# Autodesk Inventor assembly: tower_MIR
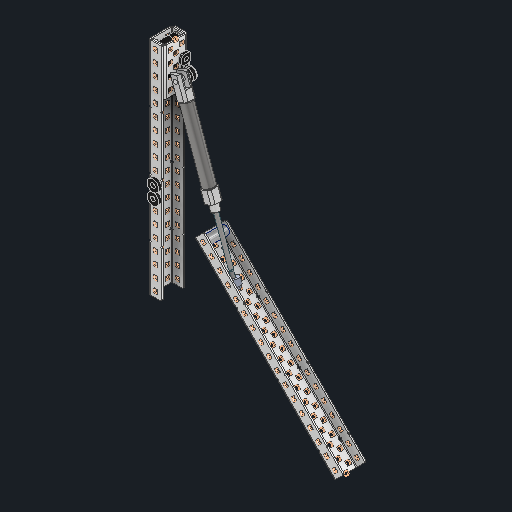
[picture p0: Inventor's stored thumbnail of the model, 512x512]
Saved by Autodesk Inventor 2024 (Build 280153000, 153)
## iProperties
Created: 2024-01-16
Part Number: tower_MIR
Document SubType Name: Assembly
Designer: Averey Ku
Author: avere
## Documents named in this file (16)
- D:\vex_robotics\hardware\cad\zoomba_v0.3\arm\tower_MIR.iam
- D:\vex_robotics\hardware\cad\zoomba_v0.3\arm\Alu C 1x2x1x19_MIR.ipt
- D:\vex_robotics\hardware\cad\zoomba_v0.3\arm\Alu C 1x2x1x4_MIR.ipt
- D:\vex_robotics\hardware\cad\VEX-CAD-Inventor-1.41\Motion\Spacers\Spacer Nylon .500 OD\NSpacer Black .500 OD x .125.ipt
- D:\vex_robotics\hardware\cad\VEX-CAD-Inventor-1.41\Motion\Spacers\Spacer Nylon .500 OD.ipt
- D:\vex_robotics\hardware\cad\zoomba_v0.3\arm\LS Pillow Bearing Block_MIR.ipt
- D:\vex_robotics\hardware\cad\VEX-CAD-Inventor-1.41\Motion\Spacers\Spacer Nylon .375 OD\NSpacer .375 OD x .250.ipt
- D:\vex_robotics\hardware\cad\VEX-CAD-Inventor-1.41\Motion\Spacers\Spacer Nylon .375 OD.ipt
- D:\vex_robotics\hardware\cad\VEX-CAD-Inventor-1.41\Motion\Spacers\Spacer Nylon .375 OD\NSpacer .375 OD x .500.ipt
- D:\vex_robotics\hardware\cad\VEX-CAD-Inventor-1.41\Motion\Spacers\Washer Steel\SWasher .375 OD x .062500.ipt
- D:\vex_robotics\hardware\cad\VEX-CAD-Inventor-1.41\Motion\Spacers\Washer Steel.ipt
- D:\vex_robotics\hardware\cad\zoomba_v0.3\arm\Double Acting Piston_MIR.iam
- D:\vex_robotics\hardware\cad\zoomba_v0.3\arm\Alu C 1x2x1x17_MIR.ipt
- D:\vex_robotics\hardware\cad\zoomba_v0.3\arm\Shaft Collar No Screw_MIR.ipt
- D:\vex_robotics\hardware\cad\zoomba_v0.3\arm\Piston Nut_MIR.ipt
- D:\vex_robotics\hardware\cad\zoomba_v0.3\arm\.375 OD Aluminum Spacer 0.875_MIR.ipt
## Components (13 placed, 12 different names)
1. Alu C 1x2x1x19_MIR:1 — Mate:1, Insert:1, Insert:4, Insert:3, Angle:1
2. Alu C 1x2x1x4_MIR:1 — Mate:1, Insert:1, Mate:2, Insert:5, Insert:8
3. NSpacer Black .500 OD x .125:1 — Insert:4
4. NSpacer Black .500 OD x .125:2 — Insert:3
5. LS Pillow Bearing Block_MIR:1 — Mate:2, Insert:5, Insert:9
6. NSpacer .375 OD x .250:1 — Insert:7, Insert:6
7. NSpacer .375 OD x .500:2 — Insert:8, Insert:7
8. SWasher .375 OD x .062500:1 — Insert:6
9. Double Acting Piston_MIR:1 [sub-assembly] — Insert:9, Insert:11
10. Alu C 1x2x1x17_MIR:1 — Angle:1, Mate:3, Insert:12
11. Shaft Collar No Screw_MIR:1 — Mate:3, Insert:10
12. Piston Nut_MIR:1 — Insert:11, Insert:10
13. .375 OD Aluminum Spacer 0.875_MIR:1 — Insert:12
## Relationships (15: Insert 11, Mate 3, Angle 1)
- Mate:1: Alu C 1x2x1x19_MIR:1 ↔ Alu C 1x2x1x4_MIR:1
- Insert:1: Alu C 1x2x1x19_MIR:1 ↔ Alu C 1x2x1x4_MIR:1
- Insert:4: Alu C 1x2x1x19_MIR:1 ↔ NSpacer Black .500 OD x .125:1
- Insert:3: Alu C 1x2x1x19_MIR:1 ↔ NSpacer Black .500 OD x .125:2
- Mate:2: Alu C 1x2x1x4_MIR:1 ↔ LS Pillow Bearing Block_MIR:1
- Insert:5 (1.5875 mm): Alu C 1x2x1x4_MIR:1 ↔ LS Pillow Bearing Block_MIR:1
- Insert:8: Alu C 1x2x1x4_MIR:1 ↔ NSpacer .375 OD x .500:2
- Insert:7: NSpacer .375 OD x .250:1 ↔ NSpacer .375 OD x .500:2
- Insert:6: NSpacer .375 OD x .250:1 ↔ SWasher .375 OD x .062500:1
- Insert:9: LS Pillow Bearing Block_MIR:1 ↔ Double Acting Piston_MIR:1
- Angle:1 (0 deg): Alu C 1x2x1x19_MIR:1 ↔ Alu C 1x2x1x17_MIR:1
- Mate:3: Alu C 1x2x1x17_MIR:1 ↔ Shaft Collar No Screw_MIR:1
- Insert:11: Double Acting Piston_MIR:1 ↔ Piston Nut_MIR:1
- Insert:10: Shaft Collar No Screw_MIR:1 ↔ Piston Nut_MIR:1
- Insert:12: Alu C 1x2x1x17_MIR:1 ↔ .375 OD Aluminum Spacer 0.875_MIR:1
